# Autodesk Inventor assembly: POM_T5_04
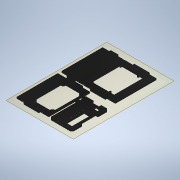
[picture p0: Inventor's stored thumbnail of the model, 180x180]
Saved by Autodesk Inventor 2020 (Build 240168000, 168)
## iProperties
Created: 2021-08-27
Part Number: POM_T5_04
Document SubType Name: Assembly
Designer: Masato
Author: Masato
## Documents named in this file (6)
- C:\Inventor\OpenPlatform_ver3_0\cam\POM_T5_04.iam
- C:\Inventor\OpenPlatform_ver3_0\cam\Disposable_Board.ipt
- C:\Inventor\OpenPlatform_ver3_0\UpperBody\Cockpit\Cockpit_bottom_frame.ipt
- C:\Inventor\OpenPlatform_ver3_0\UpperBody\Cockpit\Cockpit_front_frame.ipt
- C:\Inventor\OpenPlatform_ver3_0\UpperBody\Cockpit\Cockpit_middle_frame.ipt
- C:\Inventor\OpenPlatform_ver3_0\UpperBody\Cockpit\Cockpit_side_frame.ipt
## Components (5 placed, 5 different names)
1. Disposable_Board:1 — メイト:2, メイト:1, フラッシュ:1, フラッシュ:2, メイト:4, メイト:5, メイト:6, メイト:7, フラッシュ:3, フラッシュ:4, フラッシュ:5, フラッシュ:6
2. Cockpit_bottom_frame:1 — メイト:4, フラッシュ:3, フラッシュ:4, メイト:8, メイト:9
3. Cockpit_front_frame:1 — メイト:7, メイト:8, フラッシュ:5, フラッシュ:7, メイト:10
4. Cockpit_middle_frame:1 — メイト:5, フラッシュ:7, メイト:10
5. Cockpit_side_frame:1 — メイト:6, フラッシュ:6, メイト:9
## Relationships (16: Mate 9, Flush 7)
- メイト:2 [Mate]: Disposable_Board:1
- メイト:1 [Mate]: Disposable_Board:1
- フラッシュ:1 [Flush]: Disposable_Board:1
- フラッシュ:2 [Flush]: Disposable_Board:1
- メイト:4 [Mate]: Disposable_Board:1 ↔ Cockpit_bottom_frame:1
- メイト:5 [Mate]: Disposable_Board:1 ↔ Cockpit_middle_frame:1
- メイト:6 [Mate]: Disposable_Board:1 ↔ Cockpit_side_frame:1
- メイト:7 [Mate]: Disposable_Board:1 ↔ Cockpit_front_frame:1
- フラッシュ:3 [Flush] (2.5 mm): Disposable_Board:1 ↔ Cockpit_bottom_frame:1
- フラッシュ:4 [Flush] (2.5 mm): Disposable_Board:1 ↔ Cockpit_bottom_frame:1
- メイト:8 [Mate] (2.5 mm): Cockpit_bottom_frame:1 ↔ Cockpit_front_frame:1
- フラッシュ:5 [Flush] (2.5 mm): Disposable_Board:1 ↔ Cockpit_front_frame:1
- フラッシュ:6 [Flush] (2.5 mm): Disposable_Board:1 ↔ Cockpit_side_frame:1
- メイト:9 [Mate] (2.5 mm): Cockpit_bottom_frame:1 ↔ Cockpit_side_frame:1
- フラッシュ:7 [Flush]: Cockpit_front_frame:1 ↔ Cockpit_middle_frame:1
- メイト:10 [Mate] (2.5 mm): Cockpit_front_frame:1 ↔ Cockpit_middle_frame:1
